# Autodesk Inventor assembly: New Guard
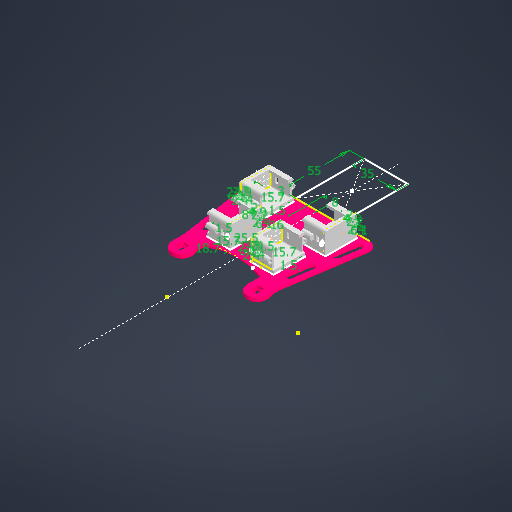
[picture p0: Inventor's stored thumbnail of the model, 512x512]
Saved by Autodesk Inventor 2026.1 (Build 301233000, 233)
## iProperties
Created: 2026-03-02
Part Number: New Guard
Document SubType Name: Assembly
Designer: sp16709
Author: sp16709
## Documents named in this file (5)
- D:\BioRobotics Inventor Files\Main Directory\New Guard.iam
- D:\BioRobotics Inventor Files\Main Directory\Arm Guard.ipt
- D:\BioRobotics Inventor Files\Main Directory\Horizontal_Servo_Adapter.ipt
- D:\BioRobotics Inventor Files\Main Directory\MG90S Servo.ipt
- C:\Users\WinFlame\Documents\Inventor\Content Center Files\R2026\en-US\AS 1427(08)\AS 1427 - M2.5 x 4(6) I.ipt
## Components (11 placed, 4 different names)
1. Arm Guard:1 — Mate:1, Mate:4, Mate:12, Mate:16, Mate:18, Mate:19, Mate:20, Mate:22, Mate:23, Mate:24, Mate:25, Mate:26, Mate:27
2. Horizontal_Servo_Adapter:1 — Mate:6, Mate:8, Mate:10, Mate:11, Mate:16, Mate:22
3. Horizontal_Servo_Adapter:2 — Mate:1, Mate:2, Mate:12, Mate:13, Mate:14, Mate:15, Mate:23
4. Horizontal_Servo_Adapter:3 — Mate:24, Mate:25, Mate:32, Mate:33, Mate:34
5. Horizontal_Servo_Adapter:4 — Mate:26, Mate:27, Mate:30, Mate:31
6. MG90S Servo:1 — Mate:8, Mate:10, Mate:11
7. MG90S Servo:2 — Mate:13, Mate:14, Mate:15
8. MG90S Servo:3 — Mate:32, Mate:33, Mate:34
9. MG90S Servo:4 — Mate:30, Mate:31, Insert:1, Insert:2
10. AS 1427 Z - Metric M2.5 x 4:1 — Insert:1
11. AS 1427 Z - Metric M2.5 x 4:2 — Insert:2
## Relationships (31: Mate 29, Insert 2)
- Mate:1: Arm Guard:1 ↔ Horizontal_Servo_Adapter:2
- Mate:2: Horizontal_Servo_Adapter:2
- Mate:4: Arm Guard:1
- Mate:5
- Mate:6: Horizontal_Servo_Adapter:1
- Mate:7
- Mate:8: Horizontal_Servo_Adapter:1 ↔ MG90S Servo:1
- Mate:10: Horizontal_Servo_Adapter:1 ↔ MG90S Servo:1
- Mate:11: Horizontal_Servo_Adapter:1 ↔ MG90S Servo:1
- Mate:12: Arm Guard:1 ↔ Horizontal_Servo_Adapter:2
- Mate:13: Horizontal_Servo_Adapter:2 ↔ MG90S Servo:2
- Mate:14: Horizontal_Servo_Adapter:2 ↔ MG90S Servo:2
- Mate:15: Horizontal_Servo_Adapter:2 ↔ MG90S Servo:2
- Mate:16: Arm Guard:1 ↔ Horizontal_Servo_Adapter:1
- Mate:18: Arm Guard:1
- Mate:19: Arm Guard:1
- Mate:20: Arm Guard:1
- Mate:21
- Mate:22: Arm Guard:1 ↔ Horizontal_Servo_Adapter:1
- Mate:23: Arm Guard:1 ↔ Horizontal_Servo_Adapter:2
- Mate:24: Arm Guard:1 ↔ Horizontal_Servo_Adapter:3
- Mate:25: Arm Guard:1 ↔ Horizontal_Servo_Adapter:3
- Mate:26: Arm Guard:1 ↔ Horizontal_Servo_Adapter:4
- Mate:27: Arm Guard:1 ↔ Horizontal_Servo_Adapter:4
- Mate:30: Horizontal_Servo_Adapter:4 ↔ MG90S Servo:4
- Mate:31: Horizontal_Servo_Adapter:4 ↔ MG90S Servo:4
- Mate:32: Horizontal_Servo_Adapter:3 ↔ MG90S Servo:3
- Mate:33: Horizontal_Servo_Adapter:3 ↔ MG90S Servo:3
- Mate:34: Horizontal_Servo_Adapter:3 ↔ MG90S Servo:3
- Insert:1: MG90S Servo:4 ↔ AS 1427 Z - Metric M2.5 x 4:1
- Insert:2: MG90S Servo:4 ↔ AS 1427 Z - Metric M2.5 x 4:2
